# Autodesk Inventor assembly: Blum_48N0510_hanging_mechanism_LR_pair_w_hook
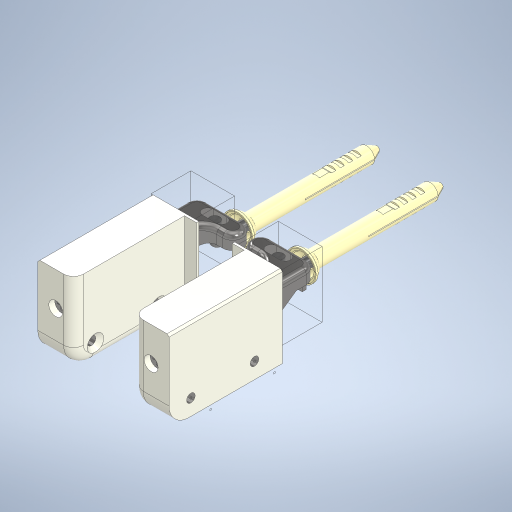
[picture p0: Inventor's stored thumbnail of the model, 512x512]
Saved by Autodesk Inventor 2024 (Build 280153000, 153)
## iProperties
Created: 2019-11-11
Part Number: Blum_48N0510_hanging_mechanism_LR_pair_w_hook
Document SubType Name: Assembly
Designer: RokasM
Author: RokasM
## Documents named in this file (6)
- C:\W4INV 2024 Design\LIBRARY\Wall hanging hardware\Blum_48N0510_hanging_mechanism\Blum_48N0510_hanging_mechanism.iam
- C:\W4INV 2024 Design\LIBRARY\Wall hanging hardware\Blum_48N0510_hanging_mechanism\Blum_48N0510_hanging_mechanism\Blum_48N0510_02_Right_w_hook.ipt
- C:\W4INV 2024 Design\LIBRARY\Wall hanging hardware\Blum_48N0510_hanging_mechanism\Blum_48N0510_hanging_mechanism.ipt
- C:\W4INV 2024 Design\LIBRARY\Wall hanging hardware\Blum_48N0510_hanging_mechanism\Blum_48N0510_hanging_mechanism\Blum_48N0510_03_Left_w_hook.ipt
- Blum_48N0510_hanging_mechanism_LR_pair_no_hook.iam
- Blum_48N0510_hanging_mechanism_LR_pair_w_hook.iam
## Components (2 placed, 2 different names)
1. Blum_48N0510_02_Right_w_hook:1 — Flush:1, Flush:2
2. Blum_48N0510_03_Left_w_hook:2 — Flush:1, Flush:2
## Relationships (2: Flush 2)
- Flush:1: Blum_48N0510_02_Right_w_hook:1 ↔ Blum_48N0510_03_Left_w_hook:2
- Flush:2: Blum_48N0510_02_Right_w_hook:1 ↔ Blum_48N0510_03_Left_w_hook:2
